# Autodesk Inventor assembly: HTD-45H Assembly
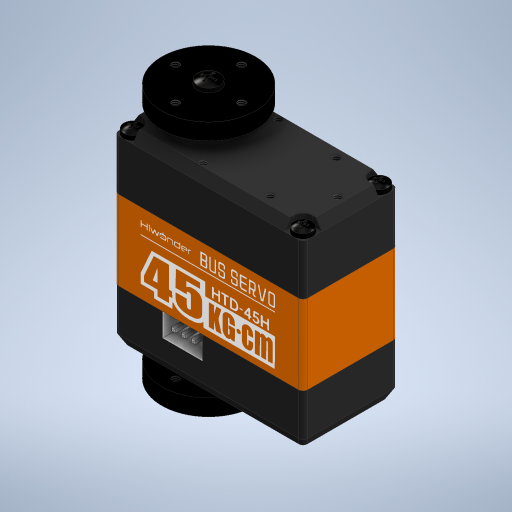
[picture p0: Inventor's stored thumbnail of the model, 512x512]
Saved by Autodesk Inventor 2024.1 (Build 281209000, 209)
## iProperties
Created: 2023-08-18
Part Number: HTD-45H Assembly
Document SubType Name: Assembly
Designer: chanh
Mass: 69.2965 g
Surface Area: 112.775 cm^2
Volume: 34.3975 cm^3
Density: 2.01458 g/cm^3
Author: chanh
## Documents named in this file (6)
- C:\Users\chanh\OneDrive - 연세대학교 (Yonsei University)\로봇\Humanoid\Roboin Humanoid Project\Inventor\rh_plus_7_axis_robot_arm_hardware\Part\HTD-45H, Horn\HTD-45H Assembly.iam
- C:\Users\chanh\OneDrive - 연세대학교 (Yonsei University)\로봇\Humanoid\Roboin Humanoid Project\Inventor\rh_plus_7_axis_robot_arm_hardware\Part\HTD-45H, Horn\HTD-45H\HTD-45H.iam
- C:\Users\chanh\OneDrive - 연세대학교 (Yonsei University)\로봇\Humanoid\Roboin Humanoid Project\Inventor\rh_plus_7_axis_robot_arm_hardware\Part\HTD-45H, Horn\Horn\Top Horn.ipt
- C:\Users\chanh\OneDrive - 연세대학교 (Yonsei University)\로봇\Humanoid\Roboin Humanoid Project\Inventor\rh_plus_7_axis_robot_arm_hardware\Part\HTD-45H, Horn\Horn\Bottom Horn.ipt
- C:\Users\chanh\OneDrive - 연세대학교 (Yonsei University)\로봇\Humanoid\Roboin Humanoid Project\Inventor\rh_plus_7_axis_robot_arm_hardware\Part\HTD-45H, Horn\Horn\M3x6.ipt
- C:\Users\chanh\OneDrive - 연세대학교 (Yonsei University)\로봇\Humanoid\Roboin Humanoid Project\Inventor\rh_plus_7_axis_robot_arm_hardware\Part\HTD-45H, Horn\Horn\M3x5.ipt
## Components (5 placed, 5 different names)
1. HTD-45H:1 [sub-assembly] — Flush:1, Flush:2, Flush:3, Rotational:1, Rotational:2
2. Top Horn:1 — Rotational:1, Rigid:1
3. Bottom Horn:1 — Rotational:2, Rigid:2
4. M3x6:1 — Rigid:1
5. M3x5:1 — Rigid:2
## Relationships (7: Flush 3, RevoluteJoint 2, WeldJoint 2)
- Flush:1: HTD-45H:1
- Flush:2: HTD-45H:1
- Flush:3: HTD-45H:1
- Rotational:1 [RevoluteJoint]: HTD-45H:1 ↔ Top Horn:1
- Rotational:2 [RevoluteJoint]: HTD-45H:1 ↔ Bottom Horn:1
- Rigid:1 [WeldJoint]: Top Horn:1 ↔ M3x6:1
- Rigid:2 [WeldJoint]: Bottom Horn:1 ↔ M3x5:1
